# Autodesk Inventor assembly: plateau_cyclique
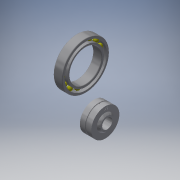
[picture p0: Inventor's stored thumbnail of the model, 180x180]
Saved by Autodesk Inventor 2018 (Build 220112000, 112)
## iProperties
Created: 2017-10-15
Part Number: plateau_cyclique
Document SubType Name: Assembly
Designer: liamg
Author: liamg
## Documents named in this file (6)
- D:\Glabs\Helicopter_v1\CAD\Rotor\plateau_cylique\plateau_cyclique.iam
- C:\Users\liamg\Desktop\plateau rotor\Rouleement a bille_PARTserver02017101500132795162595192d056f\_61805_PART1.ipt
- C:\Users\liamg\Desktop\plateau rotor\Rouleement a bille_PARTserver02017101500132795162595192d056f\_61805_PART2.ipt
- C:\Users\liamg\Desktop\plateau rotor\Rouleement a bille_PARTserver02017101500132795162595192d056f\_61805_PART3.ipt
- C:\Users\liamg\Desktop\plateau rotor\Rotule_HPC_HPCSSE845\_hpc_SSE8.45_1.ipt
- C:\Users\liamg\Desktop\plateau rotor\Rotule_HPC_HPCSSE845\_hpc_SSE8.45_2.ipt
## Components (19 placed, 7 different names)
1. Roulement_a_bille_d_int — Rotational:1
2. Roulement_a_bille_d_ext — Rotational:1
3. bille_1
4. bille_2
5. _61805_PART3:3
6. _61805_PART3:4
7. _61805_PART3:5
8. _61805_PART3:6
9. _61805_PART3:7
10. _61805_PART3:8
11. _61805_PART3:9
12. _61805_PART3:10
13. _61805_PART3:11
14. _61805_PART3:12
15. _61805_PART3:13
16. _61805_PART3:14
17. _61805_PART3:15
18. rotule_cylindre — Ball:1
19. rotule_sphere — Ball:1
## Relationships (2: BallJoint 1, RevoluteJoint 1)
- Ball:1: rotule_cylindre ↔ rotule_sphere
- Rotational:1 [RevoluteJoint]: Roulement_a_bille_d_int ↔ Roulement_a_bille_d_ext
